# Autodesk Inventor assembly: CapTop-ver1-1111-2021
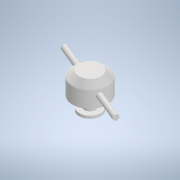
[picture p0: Inventor's stored thumbnail of the model, 180x180]
Saved by Autodesk Inventor 2021 (Build 250183000, 183)
## iProperties
Created: 2021-01-28
Part Number: CapTop-ver1-1111-2021
Document SubType Name: Assembly
Designer: con_c_000
Author: con_c_000
## Documents named in this file (3)
- F:\PHRC CADD 2021\2021 Game Design Challenge\Anchor\CapTop-ver1-1111-2021.iam
- F:\PHRC CADD 2021\2021 Game Design Challenge\Anchor\capistan lower.ipt
- F:\PHRC CADD 2021\2021 Game Design Challenge\Anchor\capistan upper.ipt
## Components (2 placed, 2 different names)
1. capistan lower:1 — Rotational:1
2. capistan upper:1 — Rotational:1
## Relationships (1: RevoluteJoint 1)
- Rotational:1 [RevoluteJoint]: capistan lower:1 ↔ capistan upper:1
